# Autodesk Inventor assembly: catapfc2
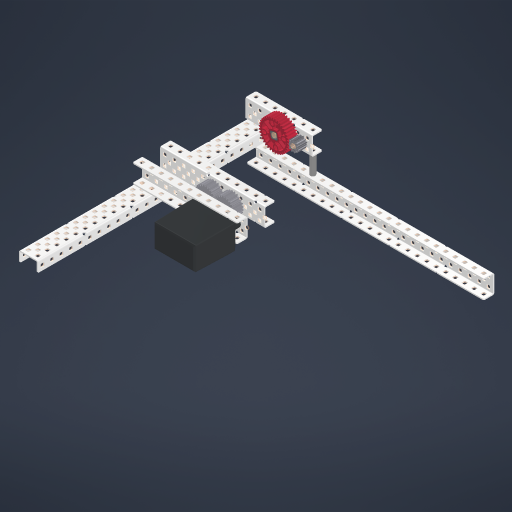
[picture p0: Inventor's stored thumbnail of the model, 512x512]
Saved by Autodesk Inventor 2024 (Build 280153000, 153)
## iProperties
Created: 2023-10-21
Part Number: catapfc2
Document SubType Name: Assembly
Designer: macbook
Author: macbook
## Documents named in this file (11)
- \\Mac\Home\Desktop\code\1599V-VRC\Cad\Assembly\v2\catapfc2.iam
- \\Mac\Home\Desktop\code\1599V-VRC\Cad\Structure\C Channel\Aluminum 1x2x1\Alu C 1x2x1x25.ipt
- \\Mac\Home\Desktop\code\1599V-VRC\Cad\Motion\Gears\HS Gear\HS 12T Gear, No Insert.iam
- \\Mac\Home\Desktop\code\1599V-VRC\Cad\Motion\Gears\HS Gear.iam
- \\Mac\Home\Desktop\code\1599V-VRC\Cad\Motion\Gears\HS Gear\HS 24T Gear, No Insert.iam
- \\Mac\Home\Desktop\code\1599V-VRC\Cad\Motion\Gears\HS Gear\HS 36T Gear, No Insert.iam
- \\Mac\Home\Desktop\code\1599V-VRC\Cad\Electronics\V5 Simple Motor.ipt
- \\Mac\Home\Desktop\code\1599V-VRC\Cad\Structure\C Channel\Aluminum 1x2x1\Alu C 1x2x1x11.ipt
- \\Mac\Home\Desktop\code\1599V-VRC\Cad\Structure\C Channel\Aluminum 1x2x1\Alu C 1x2x1x7.ipt
- \\Mac\Home\Desktop\code\1599V-VRC\Cad\Structure\Standoff\Standoff 1.00.ipt
- \\Mac\Home\Desktop\code\1599V-VRC\Cad\Structure\Standoff.ipt
## Components (11 placed, 8 different names)
1. Alu C 1x2x1x25:1 — Insert:12
2. Alu C 1x2x1x25:2 — Insert:10, Insert:11
3. HS 12T Gear, No Insert:1 [sub-assembly] — Insert:13
4. HS 24T Gear, No Insert:2 [sub-assembly]
5. HS 24T Gear, No Insert:3 [sub-assembly]
6. HS 36T Gear, No Insert:4 [sub-assembly] — Insert:14
7. V5 Simple Motor:1 — Insert:9
8. Alu C 1x2x1x11:1 — Insert:9
9. Alu C 1x2x1x11:2
10. Alu C 1x2x1x7:1 — Insert:10, Insert:11, Insert:13, Insert:14
11. Standoff 1.00:1 — Insert:12
## Relationships (14: Insert 14)
- [Insert] (25.4 mm): Alu C 1x2x1x25:1 ↔ Alu C 1x2x1x25:2
- [Insert] (25.4 mm): Alu C 1x2x1x25:1 ↔ Alu C 1x2x1x25:2
- [Insert]: Alu C 1x2x1x25:2 ↔ Alu C 1x2x1x11:1
- [Insert]: Alu C 1x2x1x25:2 ↔ Alu C 1x2x1x11:1
- [Insert]: Alu C 1x2x1x25:2 ↔ Alu C 1x2x1x11:2
- [Insert]: Alu C 1x2x1x25:2 ↔ Alu C 1x2x1x11:2
- [Insert] (6.35 mm): HS 24T Gear, No Insert:2 ↔ Alu C 1x2x1x11:1
- [Insert] (6.35 mm): HS 24T Gear, No Insert:3 ↔ Alu C 1x2x1x11:1
- Insert:9: V5 Simple Motor:1 ↔ Alu C 1x2x1x11:1
- Insert:10: Alu C 1x2x1x25:2 ↔ Alu C 1x2x1x7:1
- Insert:11: Alu C 1x2x1x25:2 ↔ Alu C 1x2x1x7:1
- Insert:12: Alu C 1x2x1x25:1 ↔ Standoff 1.00:1
- Insert:13: HS 12T Gear, No Insert:1 ↔ Alu C 1x2x1x7:1
- Insert:14: HS 36T Gear, No Insert:4 ↔ Alu C 1x2x1x7:1
